# Autodesk Inventor assembly: assy
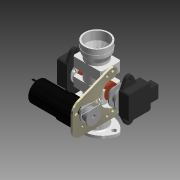
[picture p0: Inventor's stored thumbnail of the model, 180x180]
Saved by Autodesk Inventor 2015 (Build 190159000, 159)
## iProperties
Created: 2015-08-29
Part Number: assy
Document SubType Name: Assembly
Designer: francis
Author: francis
## Documents named in this file (9)
- C:\Users\francis\Documents\GitHub\CAD\assy.iam
- C:\Users\francis\Documents\GitHub\CAD\throttle_ETC.ipt
- C:\Users\francis\Documents\GitHub\CAD\bearing.ipt
- C:\Users\francis\Documents\GitHub\CAD\crouzet_motor.ipt
- C:\Users\francis\Documents\GitHub\CAD\Bosch TPS 2\Workspaces\Workspace\Bosch TPS.ipt
- C:\Users\francis\Documents\GitHub\CAD\spring_cam.ipt
- C:\Users\francis\Documents\GitHub\CAD\pulley_5mm.ipt
- C:\Users\francis\Documents\GitHub\CAD\pulley_8mm.ipt
- C:\Users\francis\Documents\GitHub\CAD\motor plate.ipt
## Components (10 placed, 8 different names)
1. throttle_ETC:1 — Mate:1, Mate:2, Mate:3, Mate:4, Mate:5, Angle:1, Angle:3, Angle:4, Symmetry:1, Angle:5, Angle:6, Angle:7, Angle:8, Flush:1, Flush:2
2. bearing:1 — Mate:2, Mate:3, Mate:6, Mate:8
3. bearing:2 — Mate:4, Mate:5, Mate:7, Mate:9
4. crouzet_motor:1 — Mate:11, Angle:6, Mate:12, Mate:14, Flush:1
5. Bosch TPS:1 — Angle:1, Mate:6
6. Bosch TPS:2 — Angle:3, Mate:7, Mate:18
7. spring_cam:1 — Mate:8, Angle:4
8. pulley_5mm:1 — Mate:14, Angle:7, Mate:16, Mate:17
9. pulley_8mm:1 — Mate:15, Angle:8, Mate:16, Mate:17
10. motor plate:1 — Flush:2, Mate:18
## Relationships (28: Mate 18, Angle 7, Flush 2, Symmetry 1)
- Mate:1: throttle_ETC:1
- Mate:2: throttle_ETC:1 ↔ bearing:1
- Mate:3: throttle_ETC:1 ↔ bearing:1
- Mate:4: throttle_ETC:1 ↔ bearing:2
- Mate:5: throttle_ETC:1 ↔ bearing:2
- Angle:1 (0 deg): throttle_ETC:1 ↔ Bosch TPS:1
- Angle:3 (180 deg): throttle_ETC:1 ↔ Bosch TPS:2
- Mate:6: bearing:1 ↔ Bosch TPS:1
- Mate:7: bearing:2 ↔ Bosch TPS:2
- Mate:8: bearing:1 ↔ spring_cam:1
- Angle:4 (0 deg): throttle_ETC:1 ↔ spring_cam:1
- Symmetry:1: throttle_ETC:1
- Mate:9: bearing:2
- Mate:10
- Angle:5 (90 deg): throttle_ETC:1
- Mate:11: crouzet_motor:1
- Angle:6 (180 deg): throttle_ETC:1 ↔ crouzet_motor:1
- Mate:12: crouzet_motor:1
- Mate:13 (48.6 mm)
- Mate:14: crouzet_motor:1 ↔ pulley_5mm:1
- Angle:7 (0 deg): throttle_ETC:1 ↔ pulley_5mm:1
- Mate:15: pulley_8mm:1
- Angle:8 (0 deg): throttle_ETC:1 ↔ pulley_8mm:1
- Mate:16: pulley_5mm:1 ↔ pulley_8mm:1
- Mate:17 (4.8527 mm): pulley_5mm:1 ↔ pulley_8mm:1
- Flush:1: throttle_ETC:1 ↔ crouzet_motor:1
- Flush:2: throttle_ETC:1 ↔ motor plate:1
- Mate:18 (22 mm): Bosch TPS:2 ↔ motor plate:1
